# Autodesk Inventor assembly: ASSEMBLY_Regolith_level_sensor_with_screws
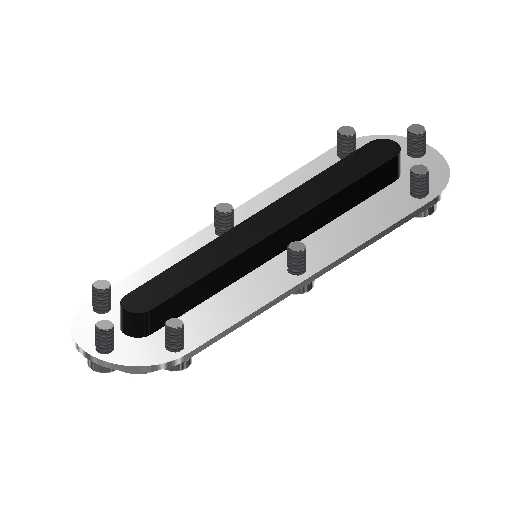
[picture p0: Inventor's stored thumbnail of the model, 512x512]
Saved by Autodesk Inventor 2025 (Build 290162010, 162A)
## iProperties
Created: 2018-09-17
Part Number: ASSEMBLY_Regolith_level_sensor_with_screws
Document SubType Name: Assembly
Designer: Andrzej
Mass: 3.54792 g
Surface Area: 16.7252 cm^2
Volume: 1.1356 cm^3
Density: 3.12427 g/cm^3
Author: Andrzej
## Documents named in this file (3)
- D:\_ANDRZEJ_LACZEWSKI\_OTHER\MECH - My entry for the NASA Lunar Sampling System Design Challenge\MCAD\1_REV1\ASSEMBLY_MAIN_REVA\ASSEMBLY_Regolith_level_sensor_with_screws.iam
- D:\_ANDRZEJ_LACZEWSKI\_OTHER\MECH - My entry for the NASA Lunar Sampling System Design Challenge\MCAD\1_REV1\ASSEMBLY_MAIN_REVA\ASSEMBLY_Regolith_level_sensor.ipt
- D:\_ANDRZEJ_LACZEWSKI\_OTHER\MECH - My entry for the NASA Lunar Sampling System Design Challenge\MCAD\1_REV1\ASSEMBLY_MAIN_REVA\CNCT_STEEL_M1,6x3_Screw.ipt
## Components (9 placed, 2 different names)
1. ASSEMBLY_Regolith_level_sensor:1 — Mate:1, Mate:2, Mate:3, Mate:4, Mate:5, Mate:6, Mate:7, Mate:8, Mate:9, Mate:10, Mate:11, Mate:12, Mate:13, Mate:14, Mate:15, Mate:16
2. CNCT_STEEL_M1,6x3_Screw:1 — Mate:7, Mate:9
3. CNCT_STEEL_M1,6x3_Screw:2 — Mate:6, Mate:11
4. CNCT_STEEL_M1,6x3_Screw:3 — Mate:1, Mate:15
5. CNCT_STEEL_M1,6x3_Screw:4 — Mate:2, Mate:14
6. CNCT_STEEL_M1,6x3_Screw:5 — Mate:5, Mate:12
7. CNCT_STEEL_M1,6x3_Screw:6 — Mate:8, Mate:10
8. CNCT_STEEL_M1,6x3_Screw:7 — Mate:3, Mate:16
9. CNCT_STEEL_M1,6x3_Screw:8 — Mate:4, Mate:13
## Relationships (16: Mate 16)
- Mate:1: ASSEMBLY_Regolith_level_sensor:1 ↔ CNCT_STEEL_M1,6x3_Screw:3
- Mate:2: ASSEMBLY_Regolith_level_sensor:1 ↔ CNCT_STEEL_M1,6x3_Screw:4
- Mate:3: ASSEMBLY_Regolith_level_sensor:1 ↔ CNCT_STEEL_M1,6x3_Screw:7
- Mate:4: ASSEMBLY_Regolith_level_sensor:1 ↔ CNCT_STEEL_M1,6x3_Screw:8
- Mate:5: ASSEMBLY_Regolith_level_sensor:1 ↔ CNCT_STEEL_M1,6x3_Screw:5
- Mate:6: ASSEMBLY_Regolith_level_sensor:1 ↔ CNCT_STEEL_M1,6x3_Screw:2
- Mate:7: ASSEMBLY_Regolith_level_sensor:1 ↔ CNCT_STEEL_M1,6x3_Screw:1
- Mate:8: ASSEMBLY_Regolith_level_sensor:1 ↔ CNCT_STEEL_M1,6x3_Screw:6
- Mate:9: ASSEMBLY_Regolith_level_sensor:1 ↔ CNCT_STEEL_M1,6x3_Screw:1
- Mate:10: ASSEMBLY_Regolith_level_sensor:1 ↔ CNCT_STEEL_M1,6x3_Screw:6
- Mate:11: ASSEMBLY_Regolith_level_sensor:1 ↔ CNCT_STEEL_M1,6x3_Screw:2
- Mate:12: ASSEMBLY_Regolith_level_sensor:1 ↔ CNCT_STEEL_M1,6x3_Screw:5
- Mate:13: ASSEMBLY_Regolith_level_sensor:1 ↔ CNCT_STEEL_M1,6x3_Screw:8
- Mate:14: ASSEMBLY_Regolith_level_sensor:1 ↔ CNCT_STEEL_M1,6x3_Screw:4
- Mate:15: ASSEMBLY_Regolith_level_sensor:1 ↔ CNCT_STEEL_M1,6x3_Screw:3
- Mate:16: ASSEMBLY_Regolith_level_sensor:1 ↔ CNCT_STEEL_M1,6x3_Screw:7
